# Autodesk Inventor assembly: Gripper
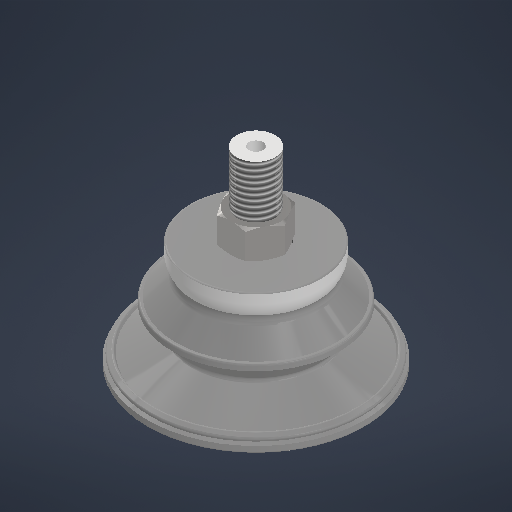
[picture p0: Inventor's stored thumbnail of the model, 512x512]
Saved by Autodesk Inventor 2026.3 (Build 303398000, 398)
## iProperties
Created: 2026-06-14
Part Number: Gripper
Document SubType Name: Assembly
Designer: ASUS
Author: ASUS
## Documents named in this file (4)
- C:\Users\ASUS\Downloads\Gripper\Gripper.iam
- C:\Users\ASUS\Downloads\Gripper\Chupaipt.ipt
- C:\Users\ASUS\Downloads\Gripper\Tuerca.ipt
- C:\Users\ASUS\Downloads\Gripper\Tornillo.ipt
## Components (3 placed, 3 different names)
1. Chupaipt:1 — Coincidencia:1, Ángulo:1, Coincidencia:2
2. Tuerca hexagonal - Pulgadas 3/8 - 16:1 — Coincidencia:1, Ángulo:1, Coincidencia:2, Coincidencia:3, Coincidencia:4
3. Tornillo:1 — Coincidencia:3, Coincidencia:4
## Relationships (5: Mate 4, Angle 1)
- Coincidencia:1 [Mate]: Chupaipt:1 ↔ Tuerca hexagonal - Pulgadas 3/8 - 16:1
- Ángulo:1 [Angle] (0 deg): Chupaipt:1 ↔ Tuerca hexagonal - Pulgadas 3/8 - 16:1
- Coincidencia:2 [Mate]: Chupaipt:1 ↔ Tuerca hexagonal - Pulgadas 3/8 - 16:1
- Coincidencia:3 [Mate]: Tuerca hexagonal - Pulgadas 3/8 - 16:1 ↔ Tornillo:1
- Coincidencia:4 [Mate]: Tuerca hexagonal - Pulgadas 3/8 - 16:1 ↔ Tornillo:1
